# Autodesk Inventor assembly: Lift bracket
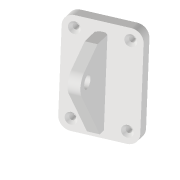
[picture p0: Inventor's stored thumbnail of the model, 180x180]
Saved by Autodesk Inventor 2020.1 (Build 241239000, 239)
## iProperties
Created: 2019-10-07
Part Number: Lift bracket
Document SubType Name: Weldment
Designer: thom_tremblay
Weld Material: Welded Aluminum-6061
Author: thom_tremblay
## Documents named in this file (3)
- C:\Users\thom_tremblay\Desktop\Inventor ACP Data\Lift bracket.iam
- C:\Users\thom_tremblay\Desktop\Inventor ACP Data\Base plate.ipt
- C:\Users\thom_tremblay\Desktop\Inventor ACP Data\Catch plate.ipt
## Components (2 placed, 2 different names)
1. Base plate:1 — Rigid:1
2. Catch plate:1 — Rigid:1
## Relationships (1: WeldJoint 1)
- Rigid:1 [WeldJoint] (-10.16 mm): Base plate:1 ↔ Catch plate:1
